# Autodesk Inventor assembly: 조립품1
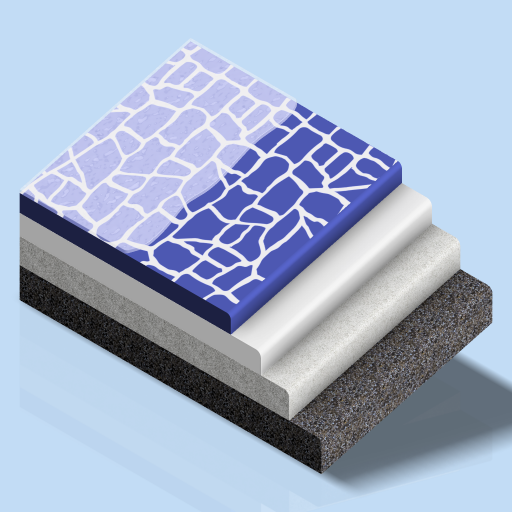
[picture p0: Inventor's stored thumbnail of the model, 512x512]
Saved by Autodesk Inventor 2024 (Build 280153000, 153)
## iProperties
Created: 2024-01-19
Part Number: 조립품1
Document SubType Name: Assembly
Designer: KBU
Author: KBU
## Documents named in this file (3)
- D:\기타\김우진\조립품1.iam
- D:\기타\김우진\유리.ipt
- D:\기타\김우진\콘크리트 제품 사진.ipt
## Components (2 placed, 2 different names)
1. 콘크리트 제품 사진:1 — 강체:1
2. 유리:1 — 강체:1
## Relationships (1: WeldJoint 1)
- 강체:1 [WeldJoint]: 콘크리트 제품 사진:1 ↔ 유리:1
